# Autodesk Inventor assembly: A2017_T4_06
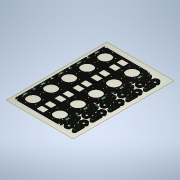
[picture p0: Inventor's stored thumbnail of the model, 180x180]
Saved by Autodesk Inventor 2022 (Build 260153000, 153)
## iProperties
Created: 2022-09-28
Part Number: A2017_T4_06
Document SubType Name: Assembly
Designer: Masato
Author: Masato
## Documents named in this file (4)
- C:\Users\ヨコオリク\Documents\CITBrains\SUSTAINA-OP\Cam\A2017_T4\A2017_T4_06.iam
- C:\Users\ヨコオリク\Documents\CITBrains\SUSTAINA-OP\Cam\DisposableBoard.ipt
- C:\Users\ヨコオリク\Documents\CITBrains\SUSTAINA-OP\LowerBody\Ankle\Ankle_side_pitch_frame.ipt
- C:\Users\ヨコオリク\Documents\CITBrains\SUSTAINA-OP\UpperBody\Trunk\Trunk_waisit_frame.ipt
## Components (16 placed, 3 different names)
1. DisposableBoard:1 — フラッシュ:1, フラッシュ:2, フラッシュ:3, フラッシュ:4, フラッシュ:5, フラッシュ:6, 正接:1, 正接:2
2. Trunk_waisit_frame:1 — メイト:1, フラッシュ:5, フラッシュ:6, メイト:3
3. Trunk_waisit_frame:2
4. Trunk_waisit_frame:3
5. Trunk_waisit_frame:4
6. Trunk_waisit_frame:5
7. Ankle_side_pitch_frame:1 — メイト:2, 正接:1, メイト:3, メイト:5
8. Ankle_side_pitch_frame:2 — メイト:4, メイト:5, 正接:2
9. Ankle_side_pitch_frame:3
10. Ankle_side_pitch_frame:4
11. Ankle_side_pitch_frame:5
12. Ankle_side_pitch_frame:6
13. Ankle_side_pitch_frame:7
14. Ankle_side_pitch_frame:8
15. Ankle_side_pitch_frame:9
16. Ankle_side_pitch_frame:10
## Component patterns: (5 elements, first: Trunk_waisit_frame:1), (5 elements, first: Ankle_side_pitch_frame:1 + Ankle_side_pitch_frame:2)
## Relationships (13: Flush 6, Mate 5, Tangent 2)
- フラッシュ:1 [Flush]: DisposableBoard:1
- フラッシュ:2 [Flush]: DisposableBoard:1
- フラッシュ:3 [Flush]: DisposableBoard:1
- フラッシュ:4 [Flush]: DisposableBoard:1
- メイト:1 [Mate]: Trunk_waisit_frame:1
- フラッシュ:5 [Flush] (2 mm): DisposableBoard:1 ↔ Trunk_waisit_frame:1
- フラッシュ:6 [Flush] (2 mm): DisposableBoard:1 ↔ Trunk_waisit_frame:1
- メイト:2 [Mate]: Ankle_side_pitch_frame:1
- 正接:1 [Tangent] (2 mm): DisposableBoard:1 ↔ Ankle_side_pitch_frame:1
- メイト:3 [Mate] (2.1 mm): Trunk_waisit_frame:1 ↔ Ankle_side_pitch_frame:1
- メイト:4 [Mate]: Ankle_side_pitch_frame:2
- メイト:5 [Mate] (2.2 mm): Ankle_side_pitch_frame:1 ↔ Ankle_side_pitch_frame:2
- 正接:2 [Tangent] (2 mm): DisposableBoard:1 ↔ Ankle_side_pitch_frame:2
